# Autodesk Inventor assembly: Hinge 1764
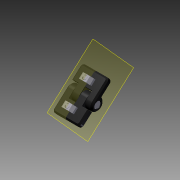
[picture p0: Inventor's stored thumbnail of the model, 180x180]
Saved by Autodesk Inventor 2011 (Build 150239000, 239)
## iProperties
Created: 2011-01-21
Part Number: Hinge 1764
Document SubType Name: Assembly
Designer: dblackburn
Author: dblackburn
## Documents named in this file (6)
- R:\2010-2011\COO\CAD\Robot 1764\Lifter 1764\Aluminum Extrusions 1764\Hinge 1764\Hinge 1764.iam
- R:\2010-2011\COO\CAD\Robot 1764\Lifter 1764\Aluminum Extrusions 1764\Hinge 1764\Hinge Screw 1764.ipt
- R:\2010-2011\COO\CAD\Robot 1764\Lifter 1764\Aluminum Extrusions 1764\Hinge 1764\Hinge Screw Bracket 1764.ipt
- R:\2010-2011\COO\CAD\Robot 1764\Lifter 1764\Aluminum Extrusions 1764\Hinge 1764\Right Hinge Plate 1764.ipt
- R:\2010-2011\COO\CAD\Robot 1764\Lifter 1764\Aluminum Extrusions 1764\Hinge 1764\Hinge Dowel 1764.ipt
- R:\2010-2011\COO\CAD\Robot 1764\Lifter 1764\Aluminum Extrusions 1764\Hinge 1764\Left Hinge Plate 1764.ipt
## Components (7 placed, 5 different names)
1. Hinge Screw Bracket 1764:1 — Insert:5, Angle:2
2. Hinge Screw 1764:2 — Insert:3, Angle:3
3. Hinge Screw Bracket 1764:2 — Insert:6, Angle:1, Mate:1
4. Hinge Screw 1764:3 — Insert:2, Angle:4
5. Right Hinge Plate 1764:1 — Insert:1, Insert:2, Insert:4, Insert:5, Angle:2, Angle:4, Angle:6
6. Hinge Dowel 1764:1 — Insert:4
7. Left Hinge Plate 1764:1 — Insert:1, Insert:3, Insert:6, Angle:1, Angle:3, Angle:6
## Relationships (13: Insert 6, Angle 6, Mate 1)
- Insert:1: Right Hinge Plate 1764:1 ↔ Left Hinge Plate 1764:1
- Insert:2: Hinge Screw 1764:3 ↔ Right Hinge Plate 1764:1
- Insert:3: Hinge Screw 1764:2 ↔ Left Hinge Plate 1764:1
- Insert:4: Right Hinge Plate 1764:1 ↔ Hinge Dowel 1764:1
- Insert:5: Hinge Screw Bracket 1764:1 ↔ Right Hinge Plate 1764:1
- Insert:6: Hinge Screw Bracket 1764:2 ↔ Left Hinge Plate 1764:1
- Angle:1 (90 deg): Hinge Screw Bracket 1764:2 ↔ Left Hinge Plate 1764:1
- Angle:2 (90 deg): Hinge Screw Bracket 1764:1 ↔ Right Hinge Plate 1764:1
- Angle:3 (0 deg): Hinge Screw 1764:2 ↔ Left Hinge Plate 1764:1
- Angle:4 (0 deg): Hinge Screw 1764:3 ↔ Right Hinge Plate 1764:1
- Mate:1: Hinge Screw Bracket 1764:2
- Angle:5 (0 deg)
- Angle:6 (0 deg): Right Hinge Plate 1764:1 ↔ Left Hinge Plate 1764:1
